# Autodesk Inventor assembly: Assembly1
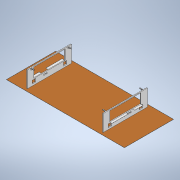
[picture p0: Inventor's stored thumbnail of the model, 180x180]
Saved by Autodesk Inventor 2021 (Build 250183000, 183)
## iProperties
Created: 2021-02-27
Part Number: Assembly1
Document SubType Name: Assembly
Designer: aidan
Author: aidan
## Documents named in this file (3)
- C:\Users\aidan\Desktop\T3 Robotics\CAD\Game Design\Assembly1.iam
- C:\Users\aidan\Desktop\T3 Robotics\CAD\Game Design\Game Design Floor.ipt
- C:\Users\aidan\Desktop\T3 Robotics\CAD\Game Design\Alliance Station.ipt
## Components (3 placed, 2 different names)
1. Game Design Floor:1 — Flush:1, Mate:1, Mate:2
2. Alliance Station:1 — Flush:1, Flush:2, Mate:2
3. Alliance Station:2 — Flush:2, Mate:1
## Relationships (4: Flush 2, Mate 2)
- Flush:1 (-457.2 mm): Game Design Floor:1 ↔ Alliance Station:1
- Flush:2: Alliance Station:1 ↔ Alliance Station:2
- Mate:1: Game Design Floor:1 ↔ Alliance Station:2
- Mate:2: Game Design Floor:1 ↔ Alliance Station:1
